# Autodesk Inventor assembly: Projeto
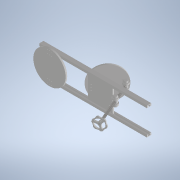
[picture p0: Inventor's stored thumbnail of the model, 180x180]
Saved by Autodesk Inventor 2021 (Build 250183000, 183)
## iProperties
Created: 2021-08-09
Part Number: Projeto
Document SubType Name: Assembly
Designer: guilh
Author: guilh
## Documents named in this file (12)
- D:\Documentos\Astronomia\Projeto Equatorial\Rail System\Rail System Project.iam
- D:\Documentos\Astronomia\Projeto Equatorial\Rail System\Tripod Base.ipt
- D:\Documentos\Astronomia\Projeto Equatorial\Rail System\Hinge.ipt
- D:\Documentos\Astronomia\Projeto Equatorial\Rail System\Moving Platform.ipt
- D:\Documentos\Astronomia\Projeto Equatorial\Rail System\Hinge Pin.ipt
- D:\Documentos\Astronomia\Projeto Equatorial\Rail System\Rail.ipt
- D:\Documentos\Astronomia\Projeto Equatorial\Rail System\Rail_Mirrored.ipt
- D:\Documentos\Astronomia\Projeto Equatorial\Rail System\Telescope Base.ipt
- D:\Documentos\Astronomia\Projeto Equatorial\Rail System\Moving Platform Pin.ipt
- D:\Documentos\Astronomia\Projeto Equatorial\Rail System\Telescope Base Pin.ipt
- D:\Documentos\Astronomia\Projeto Equatorial\Rail System\Angle Control.ipt
- D:\Documentos\Astronomia\Projeto Equatorial\Rail System\Butterfly.ipt
## Components (12 placed, 11 different names)
1. Tripod Base:1 — Mate:6, Insert:11, Insert:12
2. Hinge:1 — Mate:1, Flush:1, Insert:1, Insert:2
3. Hinge:2 — Insert:3, Mate:7, Insert:6, Insert:7
4. Moving Platform:1 — Mate:1, Flush:1, Insert:1, Mate:2, Mate:3, Mate:4, Mate:5, Insert:8
5. Hinge Pin:3 — Insert:2, Insert:3
6. Rail:1 — Flush:2, Mate:2, Mate:5, Insert:11, Insert:12
7. Rail_Mirrored:1 — Flush:2, Mate:3, Mate:4, Mate:6
8. Telescope Base:1 — Mate:7, Insert:6, Insert:7, Insert:9
9. Moving Platform Pin:1 — Insert:8, Mate:8
10. Telescope Base Pin:1 — Insert:9, Insert:10
11. Angle Control:1 — Insert:10, Mate:8, Mate:9, Mate:10, Flush:3
12. Butterfly:1 — Mate:9, Mate:10, Flush:3
## Relationships (23: Mate 10, Insert 10, Flush 3)
- Mate:1: Hinge:1 ↔ Moving Platform:1
- Flush:1: Hinge:1 ↔ Moving Platform:1
- Insert:1: Hinge:1 ↔ Moving Platform:1
- Insert:2: Hinge:1 ↔ Hinge Pin:3
- Insert:3: Hinge:2 ↔ Hinge Pin:3
- Flush:2: Rail:1 ↔ Rail_Mirrored:1
- Mate:2: Moving Platform:1 ↔ Rail:1
- Mate:3: Moving Platform:1 ↔ Rail_Mirrored:1
- Mate:4: Moving Platform:1 ↔ Rail_Mirrored:1
- Mate:5: Moving Platform:1 ↔ Rail:1
- Mate:6: Tripod Base:1 ↔ Rail_Mirrored:1
- Mate:7: Hinge:2 ↔ Telescope Base:1
- Insert:6: Hinge:2 ↔ Telescope Base:1
- Insert:7: Hinge:2 ↔ Telescope Base:1
- Insert:8 (-9 mm): Moving Platform:1 ↔ Moving Platform Pin:1
- Insert:9 (-10 mm): Telescope Base:1 ↔ Telescope Base Pin:1
- Insert:10: Telescope Base Pin:1 ↔ Angle Control:1
- Mate:8: Moving Platform Pin:1 ↔ Angle Control:1
- Mate:9: Angle Control:1 ↔ Butterfly:1
- Mate:10: Angle Control:1 ↔ Butterfly:1
- Flush:3: Angle Control:1 ↔ Butterfly:1
- Insert:11: Tripod Base:1 ↔ Rail:1
- Insert:12: Tripod Base:1 ↔ Rail:1
